# Autodesk Inventor assembly: ASM Side Drawers
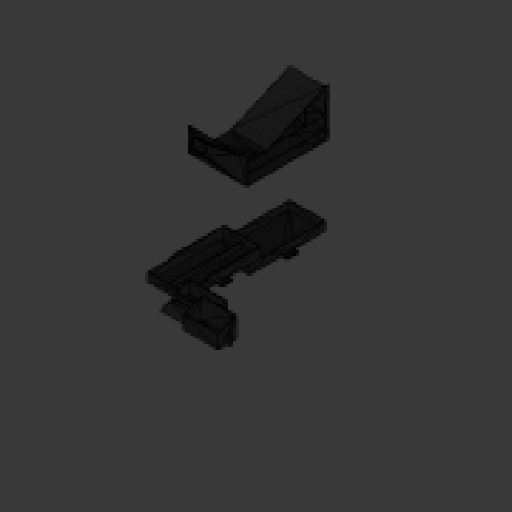
[picture p0: Inventor's stored thumbnail of the model, 512x512]
Saved by Autodesk Inventor 2023 (Build 270158000, 158)
## iProperties
Created: 2023-03-16
Part Number: ASM Side Drawers
Document SubType Name: Assembly
Designer: alber
Author: alber
## Documents named in this file (6)
- C:\Users\alber\Desktop\Files\Ender3-Upgrade\CAD\ASM Side Drawers.iam
- C:\Users\alber\Desktop\Files\Ender3-Upgrade\PCB\Ender3 Upgrade\Drawer_Bottom.ipt
- C:\Users\alber\Desktop\Files\Ender3-Upgrade\PCB\Ender3 Upgrade\Drawer_Holder.ipt
- C:\Users\alber\Desktop\Files\Ender3-Upgrade\PCB\Ender3 Upgrade\Drawer_Middle.ipt
- C:\Users\alber\Desktop\Files\Ender3-Upgrade\PCB\Ender3 Upgrade\Drawer_TopLeft.ipt
- C:\Users\alber\Desktop\Files\Ender3-Upgrade\PCB\Ender3 Upgrade\Drawer_TopRight.ipt
## Components (5 placed, 5 different names)
1. Drawer_Bottom:1 — Mate:1, Mate:2
2. Drawer_Holder:1 — Mate:1, Mate:2, Mate:3, Mate:4, Mate:5, Mate:6, Mate:7, Mate:8
3. Drawer_Middle:1 — Mate:3, Mate:4
4. Drawer_TopLeft:1 — Mate:5, Mate:6
5. Drawer_TopRight:1 — Mate:7, Mate:8
## Relationships (8: Mate 8)
- Mate:1: Drawer_Bottom:1 ↔ Drawer_Holder:1
- Mate:2: Drawer_Bottom:1 ↔ Drawer_Holder:1
- Mate:3: Drawer_Holder:1 ↔ Drawer_Middle:1
- Mate:4: Drawer_Holder:1 ↔ Drawer_Middle:1
- Mate:5: Drawer_Holder:1 ↔ Drawer_TopLeft:1
- Mate:6: Drawer_Holder:1 ↔ Drawer_TopLeft:1
- Mate:7: Drawer_Holder:1 ↔ Drawer_TopRight:1
- Mate:8: Drawer_Holder:1 ↔ Drawer_TopRight:1
